# Autodesk Inventor assembly: SoporteServo
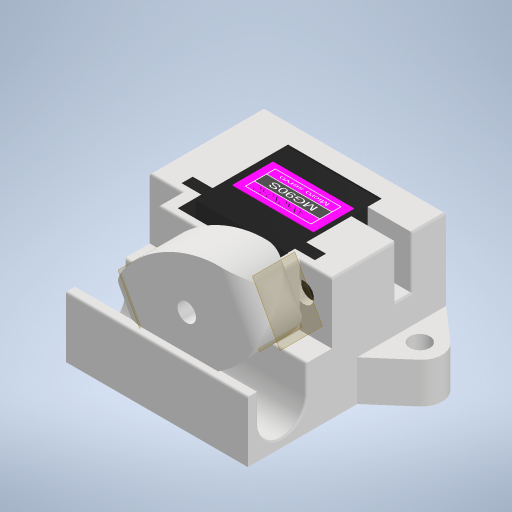
[picture p0: Inventor's stored thumbnail of the model, 512x512]
Saved by Autodesk Inventor 2024.4 (Build 284460000, 460)
## iProperties
Created: 2026-06-02
Part Number: SoporteServo
Document SubType Name: Assembly
Designer: Apleppli
Author: Apleppli
## Documents named in this file (5)
- D:\Downloads\Proyecto_POO_Pentatrikas\Base_servo\SoporteServo - copia.iam
- D:\Downloads\Proyecto_POO_Pentatrikas\Base_servo\MG90S\ServoMG90S.iam
- D:\Downloads\Proyecto_POO_Pentatrikas\Base_servo\bloqueador2XD.ipt
- D:\Downloads\Proyecto_POO_Pentatrikas\Base_servo\Bidirectional shoulder.ipt
- D:\Downloads\Proyecto_POO_Pentatrikas\Base_servo\basever2.ipt
## Components (4 placed, 4 different names)
1. basever2:1 — Mate:16, Angle:1, Mate:17
2. ServoMG90S:1 [sub-assembly] — Mate:9, Mate:15, Mate:16, Angle:1, Mate:17, Mate:20
3. bloqueador2XD:1 — Mate:9, Mate:12, Mate:13, Mate:15, Angle:2, Mate:19
4. Bidirectional shoulder:1 — Mate:12, Mate:13, Mate:19, Mate:20
## Relationships (10: Mate 8, Angle 2)
- Mate:9: ServoMG90S:1 ↔ bloqueador2XD:1
- Mate:12: bloqueador2XD:1 ↔ Bidirectional shoulder:1
- Mate:13: bloqueador2XD:1 ↔ Bidirectional shoulder:1
- Mate:15: ServoMG90S:1 ↔ bloqueador2XD:1
- Mate:16: basever2:1 ↔ ServoMG90S:1
- Angle:1 (180 deg): basever2:1 ↔ ServoMG90S:1
- Mate:17: basever2:1 ↔ ServoMG90S:1
- Angle:2 (180 deg): bloqueador2XD:1
- Mate:19: bloqueador2XD:1 ↔ Bidirectional shoulder:1
- Mate:20: ServoMG90S:1 ↔ Bidirectional shoulder:1
